# Autodesk Inventor assembly: filled_casting_tube
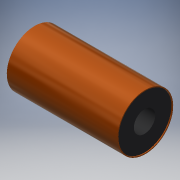
[picture p0: Inventor's stored thumbnail of the model, 180x180]
Saved by Autodesk Inventor 2017 SP1 (Build 210196100, 196)
## iProperties
Created: 2016-10-29
Part Number: filled_casting_tube
Document SubType Name: Assembly
Designer: cflannery
Author: cflannery
## Documents named in this file (3)
- D:\Triton_Rocket_Club\Propulsion\Launches\8-inch-flight\Design\CAD\Vehicle\Structures\filled_casting_tube.iam
- D:\Triton_Rocket_Club\Propulsion\Launches\8-inch-flight\Design\CAD\Vehicle\Structures\casting_tube.ipt
- D:\Triton_Rocket_Club\Propulsion\Launches\8-inch-flight\Design\CAD\Vehicle\Structures\grain.ipt
## Components (2 placed, 2 different names)
1. casting_tube:1 — Mate:1, Flush:1
2. grain:1 — Mate:1, Flush:1
## Relationships (2: Mate 1, Flush 1)
- Mate:1: casting_tube:1 ↔ grain:1
- Flush:1 (-2.54 mm): casting_tube:1 ↔ grain:1
